# Autodesk Inventor assembly: Biblow Assssssssemblee
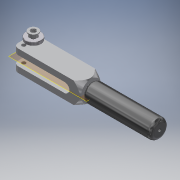
[picture p0: Inventor's stored thumbnail of the model, 180x180]
Saved by Autodesk Inventor 2017.3 (Build 213256000, 256)
## iProperties
Created: 2017-04-21
Part Number: Biblow Assssssssemblee
Document SubType Name: Assembly
Designer: 193515
Author: 193515
## Documents named in this file (11)
- C:\Users\rbibb\Desktop\8.1\Biblow Asemblee.iam
- C:\Users\193515.FCBOE.000\Documents\Part1.ipt
- C:\Users\rbibb\Desktop\8.1\handle bar.ipt
- C:\Users\rbibb\Desktop\8.1\middle handle piece (hard).ipt
- C:\Users\rbibb\Desktop\8.1\Part2.ipt
- C:\Users\rbibb\Desktop\8.1\Roller Inner Bearing.ipt
- C:\Users\rbibb\Desktop\8.1\Roller Outer Bearing.ipt
- C:\Users\rbibb\Desktop\8.1\Roller Spacer.ipt
- C:\Users\rbibb\Desktop\8.1\Roller Inner Bearing_MIR.ipt
- C:\Users\rbibb\Desktop\8.1\Roller Outer Bearing_MIR.ipt
- C:\Users\rbibb\Desktop\8.1\Roller Spacer_MIR.ipt
## Components (10 placed, 10 different names)
1. Part1:1 — Rigid:1
2. middle handle piece (hard):1 — Rigid:1, Rotational:1, Rigid:2, Flush:1
3. Part2:1 — Rotational:1, Rotational:2
4. handle bar:1 — Rotational:2
5. Roller Inner Bearing:1 — Rotational:3, Rotational:4
6. Roller Outer Bearing:1 — Rigid:2, Rotational:3
7. Roller Spacer:1 — Rotational:4
8. Roller Inner Bearing_MIR:1 — Rotational:5, Rotational:6
9. Roller Outer Bearing_MIR:1 — Rotational:5
10. Roller Spacer_MIR:1 — Rotational:6
## Relationships (9: RevoluteJoint 6, WeldJoint 2, Flush 1)
- Rigid:1 [WeldJoint]: Part1:1 ↔ middle handle piece (hard):1
- Rotational:1 [RevoluteJoint]: middle handle piece (hard):1 ↔ Part2:1
- Rotational:2 [RevoluteJoint]: Part2:1 ↔ handle bar:1
- Rigid:2 [WeldJoint]: middle handle piece (hard):1 ↔ Roller Outer Bearing:1
- Rotational:3 [RevoluteJoint]: Roller Inner Bearing:1 ↔ Roller Outer Bearing:1
- Rotational:4 [RevoluteJoint]: Roller Inner Bearing:1 ↔ Roller Spacer:1
- Flush:1 (7.9375 mm): middle handle piece (hard):1
- Rotational:5 [RevoluteJoint]: Roller Inner Bearing_MIR:1 ↔ Roller Outer Bearing_MIR:1
- Rotational:6 [RevoluteJoint]: Roller Inner Bearing_MIR:1 ↔ Roller Spacer_MIR:1
